# Autodesk Inventor assembly: Red Pump Pipe I w_ sensors v1
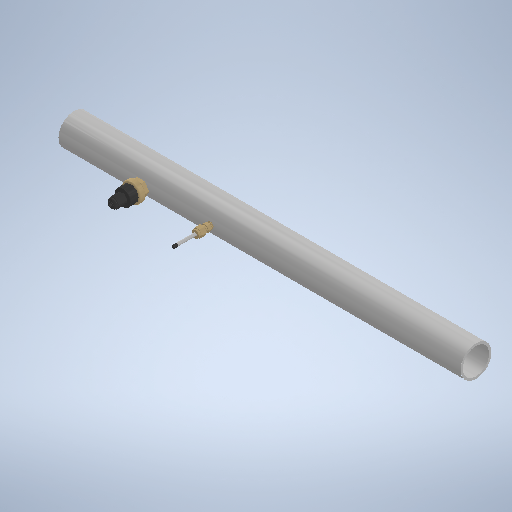
[picture p0: Inventor's stored thumbnail of the model, 512x512]
Saved by Autodesk Inventor 2027 (Build 310192000, 192)
## iProperties
Created: 2026-07-30
Part Number: Red Pump Pipe I w_ sensors v1
Document SubType Name: Assembly
Designer: AdminForWorker
Title: Pipe I w/ sensors v1
Author: AdminForWorker
## Documents named in this file (4)
- C:\Users\ig2\Desktop\SMR Thermal\thermal-loop\resources\v0.1.2\CAD\Inventor\aa FINAL MODEL with proportional valve\Red Pump Pipe I w_ sensors v1.iam
- C:\Users\ig2\Desktop\SMR Thermal\thermal-loop\resources\v0.1.2\CAD\Inventor\aa FINAL MODEL with proportional valve\Red Pump Pipe I v4.ipt
- C:\Users\ig2\Desktop\SMR Thermal\thermal-loop\resources\v0.1.2\CAD\Inventor\aa FINAL MODEL with proportional valve\Red Pump New Thermal Couple Complete v2_1.iam
- C:\Users\ig2\Desktop\SMR Thermal\thermal-loop\resources\v0.1.2\CAD\Inventor\aa FINAL MODEL with proportional valve\Red Pump 0-200 PSI transducers v1.ipt
## Components (3 placed, 3 different names)
1. Red Pump Pipe I v4:1 — Rigid:1, Rigid:2
2. Red Pump New Thermal Couple Complete v2_1:1 [sub-assembly] — Rigid:1
3. Red Pump 0-200 PSI transducers v1:1 — Rigid:2
## Relationships (2: WeldJoint 2)
- Rigid:1 [WeldJoint] (-12.7 mm): Red Pump Pipe I v4:1 ↔ Red Pump New Thermal Couple Complete v2_1:1
- Rigid:2 [WeldJoint] (-12.7 mm): Red Pump Pipe I v4:1 ↔ Red Pump 0-200 PSI transducers v1:1
